# Autodesk Inventor assembly: SAFRS-A-0001
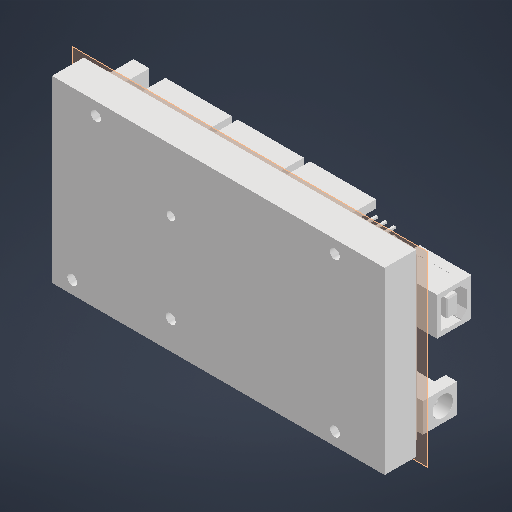
[picture p0: Inventor's stored thumbnail of the model, 512x512]
Saved by Autodesk Inventor 2026.2 (Build 302298000, 298)
## iProperties
Created: 2025-11-26
Part Number: SAFRS-A-0001
Document SubType Name: Assembly
Designer: jaewook
Author: jaewook
Title: Arduino Mega Assembly
## Documents named in this file (3)
- C:\Users\jk000\OneDrive\Desktop\git\SAFRS\mechanical\inventor\02__subassemblies\arduino_mega.iam
- C:\Users\jk000\OneDrive\Desktop\git\SAFRS\mechanical\inventor\01_parts\arduino_mega2560_step.ipt
- C:\Users\jk000\OneDrive\Desktop\git\SAFRS\mechanical\inventor\01_parts\mega_base.ipt
## Components (2 placed, 2 different names)
1. arduino_mega2560_step:1 — 플러쉬:1, 플러쉬:2
2. mega_base:1 — 플러쉬:1, 플러쉬:2
## Relationships (2: Flush 2)
- 플러쉬:1 [Flush]: arduino_mega2560_step:1 ↔ mega_base:1
- 플러쉬:2 [Flush]: arduino_mega2560_step:1 ↔ mega_base:1
